# Autodesk Inventor assembly: SRS12M1SS7907.500000
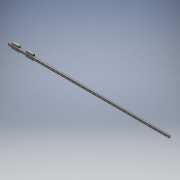
[picture p0: Inventor's stored thumbnail of the model, 180x180]
Saved by Autodesk Inventor 2016 (Build 200138000, 138)
## iProperties
Category: PARTsolutions
Company: THK
Created: 2015-05-12
Part Number: SRS12M1SS7907.500000
Catalog Web Link: www.cadenas.de
Description: Compact Type SRS-S/M/N-
Vendor: THK
Document SubType Name: Assembly
Designer: PARTuser1
Manufacturer: THK
PSOL_IDENT_0: {$CADENAS_DATA\23d-libs\thk\linear_motion_systems\lm_guide\lm_caged_ball_roller\caged_ball\lm_guide_
PSOL_IDENT_1: srs\com_typ_srs_s_m_n.prj},247 {VTYP=3D},{STYP=ASSTAB},{NB=SRS12M1SS7907.500000},{LINA=SRS12 M SS+79
PSOL_IDENT_2: 0L},{NN=Compact Type SRS-S/M/N},{DATE=04.12.2014 07:19:00},{GEOMDATE=04.12.2014 07:18:57},{VERSION=}
PSOL_IDENT_3: ,{LINEID=120},{LINESUBID=-1},{WBVAR=NOB,QZ,SO,L,G,GX,NR,POR,GPJ,P1,P2,P3,P4}  {NB=SRS12M1SS7907.5000
PSOL_IDENT_4: 00},{LINA=SRS12 M SS+790L},{KT=DUMMY},{MN=SRS12M},{LX1=70.0},{ND=3.000},{NOB=1},{QZ=},{SO=SS},{L=790
PSOL_IDENT_5: .0},{G=},{INFO=Infotext},{SO1='SS','SS- With end seals, side seals','UU','UU- With end seals (on bot
PSOL_IDENT_6: h ends)','SSHH','SSHH- With end seals, side seals and LaCS'},{LX=34.4},{EX=0},{LLL=34.4},{L0=34.4},{
PSOL_IDENT_7: LMIN=35.4},{LMINX=35.4},{GG='', 'Symmetrical (G1=G2)', 'A', 'Asymmetrical'},{GX=7.5},{GX2=7.5},{GX1=
PSOL_IDENT_8: 7.5},{RC1=No connection},{NR=},{POR=0},{POR1=0,[0:0]},{GPJ=},{INFO1=Infotext},{P1=0},{P2=0},{P3=0},{
PSOL_IDENT_9: P4=0},{LEND=3885.00},{LPORM=37.00},{LPORX=1000.00},{GPJ1='', 'None'},{PSM1=0},{PSM2=0},{PSM3=0},{PSM
PSOL_IDENT_10: 4=0},{PS1=755.6},{PS2=0},{PS3=0},{PS4=0},{PSX2=0},{PSX3=0},{PSX4=0},{M=13.00},{W=27.00},{LTR=34.40},
PSOL_IDENT_11: {B=20.00},{C=15.00},{H=3.00},{L1=20.60},{T=5.70},{K=11.00},{N=3.00},{W1=12.00},{W2=7.50},{M1=7.50},{
PSOL_IDENT_12: F=25.00},{D1=3.50},{D2=6.00},{HM=4.50},{MAXL=1340.00},{GMIN=4},{GMX=7.5},{GMAX1=31.28},{G1=5.75},{G2=
PSOL_IDENT_13: 5.75},{NX=1},{LT=1295.00},{A=32},{LF=793.25},{LM=790},{LL=786.75},{AA=31.1},{GA=10.00},{GMAX=11},{H3=
PSOL_IDENT_14: 2.00},{ON=SRS12 M},{ON1= },{L4=0},{QZ1='', 'No', 'QZ', 'Yes'},{X=1},{PPATH=srs_m/srs_m_asmtpl.prj},{
PSOL_IDENT_15: NOBX=},{INFOX=block1_1_},{INFOX2=dim_},{LX11=70.0}
SUPPLIER: THK
ARTICLENO: SRS12M1SS7907.500000
BOMINFO: SRS12 M SS+790L
CREATOR: CADENAS GmbH
Title: SRS12 M SS+790L
Author: Cadenas PARTsolutions
## Documents named in this file (3)
- C:\Users\as\Documents\Inventor\mintplacer-export\SRS12M1SS7907_500000.iam
- C:\Users\as\Documents\Inventor\mintplacer-export\SRS12M7907_5_Track.ipt
- C:\Users\as\Documents\Inventor\mintplacer-export\SRS12MSS_Slider.ipt
## Components (3 placed, 2 different names)
1. SRS12M7907_5_Track:1 — Slider:1
2. SRS12MSS_Slider:1 — Slider:1
3. SRS12MSS_Slider:2
## Component patterns: (2 elements, first: SRS12MSS_Slider:1)
## Relationships (1: TranslationJoint 1)
- Slider:1 [TranslationJoint]: SRS12M7907_5_Track:1 ↔ SRS12MSS_Slider:1
